# Autodesk Inventor assembly: ARM_036_TopandBottomRollers
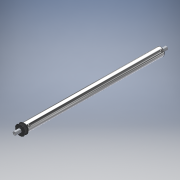
[picture p0: Inventor's stored thumbnail of the model, 180x180]
Saved by Autodesk Inventor 2018.3 (Build 223284000, 284)
## iProperties
Created: 2020-02-08
Part Number: ARM_036_TopandBottomRollers
Document SubType Name: Assembly
Designer: 22turnmaxw
Mass: 304.474 g
Surface Area: 1325.64 cm^2
Volume: 125.504 cm^3
Density: 2.42601 g/cm^3
Author: 22turnmaxw
## Documents named in this file (8)
- C:\Users\22barlalex\Documents\GrabCAD\Infinite Recharge 2020\Build season\ARM_036_TopandBottomRollers.iam
- C:\Users\22barlalex\Documents\GrabCAD\Infinite Recharge 2020\Build season\ARM_035_TopandBottomRollerTube.ipt
- C:\Users\22barlalex\Documents\GrabCAD\Infinite Recharge 2020\Build season\ARM_015_VersaRoller_Hub_1_2_Hex_Bore_x_1-1_8_OD_Aluminum_217-5895.ipt
- C:\Users\22barlalex\Documents\GrabCAD\Infinite Recharge 2020\Build season\ARM_034_36Tx9mm3mmPitchPulley.ipt
- C:\Users\22barlalex\Documents\GrabCAD\Infinite Recharge 2020\Build season\ARM_027_ANSI B18.3 - 5_16-18 UNC - UNC - 0.5.ipt
- C:\Users\22barlalex\Documents\GrabCAD\Infinite Recharge 2020\Build season\ARM_028_ANSI B18.3 - 10-24 UNC - UNC - 0.1875.ipt
- C:\Users\22barlalex\Documents\GrabCAD\Infinite Recharge 2020\Build season\ARM_055_MiddleRollerRightHexInsert.ipt
- C:\Users\22barlalex\Documents\GrabCAD\Infinite Recharge 2020\Build season\ARM_080_TopLeftHexInsert.ipt
## Components (12 placed, 7 different names)
1. ARM_035_TopandBottomRollerTube:1 — Mate:1, Mate:2, Mate:3, Mate:4, Mate:24, Mate:29, Mate:30, Mate:31, Mate:32, Tangent:1, Tangent:2, Tangent:3, Tangent:4, Rotation:1, Mate:34, Mate:41, Mate:43, Mate:49
2. ARM_015_VersaRoller_Hub_1_2_Hex_Bore_x_1-1_8_OD_Aluminum_217-5895:1 — Mate:1, Mate:2, Mate:24, Mate:52
3. ARM_015_VersaRoller_Hub_1_2_Hex_Bore_x_1-1_8_OD_Aluminum_217-5895:2 — Mate:3, Mate:4, Mate:48
4. ARM_034_36Tx9mm3mmPitchPulley:1 — Rotation:1, Mate:34, Mate:53
5. Hexagon Socket Button Head Cap Screw - Inch 5/16 - 18 x 1/2:2 — Mate:41, Mate:50, Mate:51
6. Hexagon Socket Button Head Cap Screw - Inch 10 - 24 x 3/16:1 — Mate:32, Tangent:2
7. Hexagon Socket Button Head Cap Screw - Inch 10 - 24 x 3/16:2 — Mate:29, Tangent:3
8. Hexagon Socket Button Head Cap Screw - Inch 10 - 24 x 3/16:3 — Mate:31, Tangent:1
9. Hexagon Socket Button Head Cap Screw - Inch 10 - 24 x 3/16:4 — Mate:30, Tangent:4
10. Hexagon Socket Button Head Cap Screw - Inch 5/16 - 18 x 1/2:3 — Mate:43, Mate:47
11. ARM_055_MiddleRollerRightHexInsert:2 — Mate:47, Mate:48, Mate:49
12. ARM_080_TopLeftHexInsert:1 — Mate:50, Mate:51, Mate:52, Mate:53
## Relationships (24: Mate 19, Tangent 4, RelateRotation 1)
- Mate:1: ARM_035_TopandBottomRollerTube:1 ↔ ARM_015_VersaRoller_Hub_1_2_Hex_Bore_x_1-1_8_OD_Aluminum_217-5895:1
- Mate:2: ARM_035_TopandBottomRollerTube:1 ↔ ARM_015_VersaRoller_Hub_1_2_Hex_Bore_x_1-1_8_OD_Aluminum_217-5895:1
- Mate:3: ARM_035_TopandBottomRollerTube:1 ↔ ARM_015_VersaRoller_Hub_1_2_Hex_Bore_x_1-1_8_OD_Aluminum_217-5895:2
- Mate:4: ARM_035_TopandBottomRollerTube:1 ↔ ARM_015_VersaRoller_Hub_1_2_Hex_Bore_x_1-1_8_OD_Aluminum_217-5895:2
- Mate:24: ARM_035_TopandBottomRollerTube:1 ↔ ARM_015_VersaRoller_Hub_1_2_Hex_Bore_x_1-1_8_OD_Aluminum_217-5895:1
- Mate:29: ARM_035_TopandBottomRollerTube:1 ↔ Hexagon Socket Button Head Cap Screw - Inch 10 - 24 x 3/16:2
- Mate:30: ARM_035_TopandBottomRollerTube:1 ↔ Hexagon Socket Button Head Cap Screw - Inch 10 - 24 x 3/16:4
- Mate:31: ARM_035_TopandBottomRollerTube:1 ↔ Hexagon Socket Button Head Cap Screw - Inch 10 - 24 x 3/16:3
- Mate:32: ARM_035_TopandBottomRollerTube:1 ↔ Hexagon Socket Button Head Cap Screw - Inch 10 - 24 x 3/16:1
- Tangent:1: ARM_035_TopandBottomRollerTube:1 ↔ Hexagon Socket Button Head Cap Screw - Inch 10 - 24 x 3/16:3
- Tangent:2: ARM_035_TopandBottomRollerTube:1 ↔ Hexagon Socket Button Head Cap Screw - Inch 10 - 24 x 3/16:1
- Tangent:3: ARM_035_TopandBottomRollerTube:1 ↔ Hexagon Socket Button Head Cap Screw - Inch 10 - 24 x 3/16:2
- Tangent:4: ARM_035_TopandBottomRollerTube:1 ↔ Hexagon Socket Button Head Cap Screw - Inch 10 - 24 x 3/16:4
- Rotation:1 [RelateRotation] (1.228 ul): ARM_035_TopandBottomRollerTube:1 ↔ ARM_034_36Tx9mm3mmPitchPulley:1
- Mate:34: ARM_035_TopandBottomRollerTube:1 ↔ ARM_034_36Tx9mm3mmPitchPulley:1
- Mate:41: ARM_035_TopandBottomRollerTube:1 ↔ Hexagon Socket Button Head Cap Screw - Inch 5/16 - 18 x 1/2:2
- Mate:43: ARM_035_TopandBottomRollerTube:1 ↔ Hexagon Socket Button Head Cap Screw - Inch 5/16 - 18 x 1/2:3
- Mate:47: Hexagon Socket Button Head Cap Screw - Inch 5/16 - 18 x 1/2:3 ↔ ARM_055_MiddleRollerRightHexInsert:2
- Mate:48: ARM_015_VersaRoller_Hub_1_2_Hex_Bore_x_1-1_8_OD_Aluminum_217-5895:2 ↔ ARM_055_MiddleRollerRightHexInsert:2
- Mate:49: ARM_035_TopandBottomRollerTube:1 ↔ ARM_055_MiddleRollerRightHexInsert:2
- Mate:50: Hexagon Socket Button Head Cap Screw - Inch 5/16 - 18 x 1/2:2 ↔ ARM_080_TopLeftHexInsert:1
- Mate:51: Hexagon Socket Button Head Cap Screw - Inch 5/16 - 18 x 1/2:2 ↔ ARM_080_TopLeftHexInsert:1
- Mate:52: ARM_015_VersaRoller_Hub_1_2_Hex_Bore_x_1-1_8_OD_Aluminum_217-5895:1 ↔ ARM_080_TopLeftHexInsert:1
- Mate:53: ARM_034_36Tx9mm3mmPitchPulley:1 ↔ ARM_080_TopLeftHexInsert:1
